# Autodesk Inventor assembly: S24x2
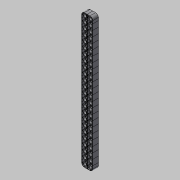
[picture p0: Inventor's stored thumbnail of the model, 180x180]
Saved by Autodesk Inventor 2020 (Build 240168000, 168)
## iProperties
Created: 2019-04-29
Part Number: S24x2
Document SubType Name: Assembly
Designer: Varga Daniel
Author: Varga Daniel
## Documents named in this file (4)
- C:\!_Dani\!_cloud\OneDrive\!_munka\Revolution\StructuralParts\Beams\Straight Beams\S2+x2\S24x2.iam
- C:\!_Dani\!_cloud\OneDrive\!_munka\Revolution\StructuralParts\Beams\beam_corner_part.ipt
- C:\!_Dani\!_cloud\OneDrive\!_munka\Revolution\StructuralParts\Beams\beam_side_part.ipt
- C:\!_Dani\!_cloud\OneDrive\!_munka\Revolution\StructuralParts\Beams\Straight Beams\S2+x2.iam
## Components (48 placed, 2 different names)
1. beam_corner_part:1 — Flush:1, Flush:2, Flush:3, Mate:1, Flush:4, Flush:5, Mate:5, Flush:12, Flush:13
2. beam_corner_part:2 — Mate:1, Flush:4, Flush:5, Corner_part_displacement, Flush:8, Flush:9
3. beam_corner_part:3 — Mate:2, Flush:6, Flush:7, Flush:8, Flush:9
4. beam_corner_part:4 — Mate:2, Flush:6, Flush:7, Corner_part_displacement
5. beam_side_part:2 — Mate:4, Flush:10, Flush:11, Mate:5
6. beam_side_part:1 — Mate:4, Flush:10, Flush:11, Flush:12, Flush:13
7. beam_side_part:3
8. beam_side_part:4
9. beam_side_part:5
10. beam_side_part:6
11. beam_side_part:7
12. beam_side_part:8
13. beam_side_part:9
14. beam_side_part:10
15. beam_side_part:11
16. beam_side_part:12
17. beam_side_part:13
18. beam_side_part:14
19. beam_side_part:15
20. beam_side_part:16
21. beam_side_part:17
22. beam_side_part:18
23. beam_side_part:19
24. beam_side_part:20
25. beam_side_part:21
26. beam_side_part:22
27. beam_side_part:23
28. beam_side_part:24
29. beam_side_part:25
30. beam_side_part:26
31. beam_side_part:27
32. beam_side_part:28
33. beam_side_part:29
34. beam_side_part:30
35. beam_side_part:31
36. beam_side_part:32
37. beam_side_part:33
38. beam_side_part:34
39. beam_side_part:35
40. beam_side_part:36
41. beam_side_part:37
42. beam_side_part:38
43. beam_side_part:39
44. beam_side_part:40
45. beam_side_part:41
46. beam_side_part:42
47. beam_side_part:43
48. beam_side_part:44
## Component patterns: (22 elements, first: beam_side_part:2 + beam_side_part:1)
## Relationships (18: Flush 13, Mate 5)
- Flush:1: beam_corner_part:1
- Flush:2: beam_corner_part:1
- Flush:3: beam_corner_part:1
- Mate:1: beam_corner_part:1 ↔ beam_corner_part:2
- Flush:4: beam_corner_part:1 ↔ beam_corner_part:2
- Flush:5: beam_corner_part:1 ↔ beam_corner_part:2
- Mate:2: beam_corner_part:3 ↔ beam_corner_part:4
- Flush:6: beam_corner_part:3 ↔ beam_corner_part:4
- Flush:7: beam_corner_part:3 ↔ beam_corner_part:4
- Corner_part_displacement [Mate] (220 mm): beam_corner_part:2 ↔ beam_corner_part:4
- Flush:8: beam_corner_part:2 ↔ beam_corner_part:3
- Flush:9: beam_corner_part:2 ↔ beam_corner_part:3
- Mate:4: beam_side_part:2 ↔ beam_side_part:1
- Flush:10: beam_side_part:2 ↔ beam_side_part:1
- Flush:11: beam_side_part:2 ↔ beam_side_part:1
- Mate:5: beam_corner_part:1 ↔ beam_side_part:2
- Flush:12: beam_corner_part:1 ↔ beam_side_part:1
- Flush:13: beam_corner_part:1 ↔ beam_side_part:1
